# Autodesk Inventor assembly: Tire
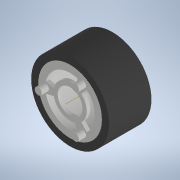
[picture p0: Inventor's stored thumbnail of the model, 180x180]
Saved by Autodesk Inventor 2022 (Build 260153000, 153)
## iProperties
Created: 2021-09-23
Part Number: Tire
Document SubType Name: Assembly
Designer: shiok
Author: shiok
## Documents named in this file (4)
- C:\Users\shiok\Documents\GitHub\Murakumo\inventor\Tire.iam
- C:\Users\shiok\Documents\GitHub\Murakumo\inventor\wheel.ipt
- C:\Users\shiok\Documents\GitHub\Murakumo\inventor\wheelcap.ipt
- C:\Users\shiok\Documents\GitHub\Murakumo\inventor\Tire.ipt
## Components (3 placed, 3 different names)
1. wheel:1 — 挿入:1, 挿入:2
2. wheelcap:1 — 挿入:1
3. Tire:1 — 挿入:2
## Relationships (2: Insert 2)
- 挿入:1 [Insert]: wheel:1 ↔ wheelcap:1
- 挿入:2 [Insert]: wheel:1 ↔ Tire:1
